# Autodesk Inventor assembly: UpperBackLink
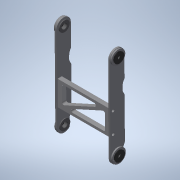
[picture p0: Inventor's stored thumbnail of the model, 180x180]
Saved by Autodesk Inventor 2020.4 (Build 244396000, 396)
## iProperties
Created: 2016-08-23
Part Number: UpperBackLink
Material: 一般
Document SubType Name: Assembly
Designer: hiro
Mass: 25.265 g
Surface Area: 146.992 cm^2
Volume: 11.3922 cm^3
Density: 2.21774 g/cm^3
Author: hiro
## Documents named in this file (6)
- C:\Users\Masato\Documents\Inventor\CIT Brains_Inventor\名称変更\OpenPlatform_ver3_0\LowerBody\リンク\UpperBackLink.iam
- C:\Users\Masato\Documents\Inventor\CIT Brains_Inventor\名称変更\OpenPlatform_ver3_0\LowerBody\リンク\Link_back_side_frame.ipt
- C:\Users\Masato\Documents\Inventor\CIT Brains_Inventor\名称変更\OpenPlatform_ver3_0\LowerBody\リンク\Link_back_diagonal.ipt
- C:\Users\Masato\Documents\Inventor\CIT Brains_Inventor\名称変更\OpenPlatform_ver3_0\Ready_Made\UUW-0312-10BH.ipt
- C:\Users\Masato\Documents\Inventor\CIT Brains_Inventor\名称変更\OpenPlatform_ver3_0\Ready_Made\80F-0603.ipt
- C:\Users\Masato\Documents\Inventor\CIT Brains_Inventor\名称変更\OpenPlatform_ver3_0\Ready_Made\LFW-0815.ipt
## Components (15 placed, 5 different names)
1. Link_back_side_frame:1 — 挿入:21, 挿入:22, 挿入:27, 挿入:28, 挿入:33, 挿入:34
2. Link_back_side_frame:2 — 挿入:23, 挿入:24, 挿入:25, 挿入:26, 挿入:35, 挿入:36
3. UUW-0312-10BH:1 — 挿入:29
4. UUW-0312-10BH:2 — 挿入:30
5. UUW-0312-10BH:3 — 挿入:31
6. UUW-0312-10BH:4 — 挿入:32
7. Link_back_diagonal:1 — 挿入:21, 挿入:22, 挿入:23, 挿入:24
8. 80F-0603:1 — 挿入:25
9. 80F-0603:2 — 挿入:26
10. 80F-0603:3 — 挿入:27
11. 80F-0603:4 — 挿入:28
12. LFW-0815:1 — 挿入:32, 挿入:35
13. LFW-0815:2 — 挿入:31, 挿入:36
14. LFW-0815:3 — 挿入:30, 挿入:33
15. LFW-0815:4 — 挿入:29, 挿入:34
## Relationships (16: Insert 16)
- 挿入:21 [Insert]: Link_back_side_frame:1 ↔ Link_back_diagonal:1
- 挿入:22 [Insert]: Link_back_side_frame:1 ↔ Link_back_diagonal:1
- 挿入:23 [Insert]: Link_back_side_frame:2 ↔ Link_back_diagonal:1
- 挿入:24 [Insert]: Link_back_side_frame:2 ↔ Link_back_diagonal:1
- 挿入:25 [Insert]: Link_back_side_frame:2 ↔ 80F-0603:1
- 挿入:26 [Insert]: Link_back_side_frame:2 ↔ 80F-0603:2
- 挿入:27 [Insert]: Link_back_side_frame:1 ↔ 80F-0603:3
- 挿入:28 [Insert]: Link_back_side_frame:1 ↔ 80F-0603:4
- 挿入:29 [Insert]: UUW-0312-10BH:1 ↔ LFW-0815:4
- 挿入:30 [Insert]: UUW-0312-10BH:2 ↔ LFW-0815:3
- 挿入:31 [Insert]: UUW-0312-10BH:3 ↔ LFW-0815:2
- 挿入:32 [Insert]: UUW-0312-10BH:4 ↔ LFW-0815:1
- 挿入:33 [Insert]: Link_back_side_frame:1 ↔ LFW-0815:3
- 挿入:34 [Insert]: Link_back_side_frame:1 ↔ LFW-0815:4
- 挿入:35 [Insert]: Link_back_side_frame:2 ↔ LFW-0815:1
- 挿入:36 [Insert]: Link_back_side_frame:2 ↔ LFW-0815:2
